# Autodesk Inventor assembly: PCBAssembly
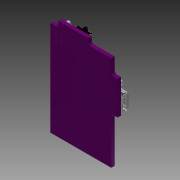
[picture p0: Inventor's stored thumbnail of the model, 180x180]
Saved by Autodesk Inventor 2015 SP2 (Build 190223200, 223)
## iProperties
Created: 2016-07-20
Part Number: PCBAssembly
Document SubType Name: Assembly
Designer: Iain
Author: Iain
## Documents named in this file (6)
- D:\Sit-To-Stand\BLEVibrator\Hardware\Case\PCBAssembly.iam
- D:\Sit-To-Stand\BLEVibrator\Hardware\Case\BarePCB.ipt
- D:\Sit-To-Stand\BLEVibrator\Hardware\Case\10118192C_USBHeader.ipt
- D:\Sit-To-Stand\BLEVibrator\Hardware\Case\RFDuino.ipt
- D:\Sit-To-Stand\BLEVibrator\Hardware\Case\SSSS810701_SlideSwitch.ipt
- D:\Sit-To-Stand\BLEVibrator\Hardware\Case\SM1204XXX_LED.ipt
## Components (6 placed, 5 different names)
1. BarePCB:1 — Mate:1, Mate:2, Flush:2, Flush:3, Mate:3, Mate:4, Flush:4, Flush:5, Flush:6, Mate:5, Mate:6, Flush:7, Flush:8, Flush:9, Flush:10
2. 10118192C_USBHeader:1 — Mate:3, Mate:4, Flush:4
3. RFDuino:1 — Mate:1, Flush:2, Flush:3
4. SSSS810701_SlideSwitch:1 — Mate:2, Flush:5, Flush:6
5. SM1204XXX_LED:1 — Mate:6, Flush:9, Flush:10
6. SM1204XXX_LED:2 — Mate:5, Flush:7, Flush:8
## Relationships (15: Flush 9, Mate 6)
- Mate:1: BarePCB:1 ↔ RFDuino:1
- Mate:2: BarePCB:1 ↔ SSSS810701_SlideSwitch:1
- Flush:2 (3.6 mm): BarePCB:1 ↔ RFDuino:1
- Flush:3 (2.2 mm): BarePCB:1 ↔ RFDuino:1
- Mate:3 (0.5 mm): BarePCB:1 ↔ 10118192C_USBHeader:1
- Mate:4 (-1.6 mm): BarePCB:1 ↔ 10118192C_USBHeader:1
- Flush:4: BarePCB:1 ↔ 10118192C_USBHeader:1
- Flush:5: BarePCB:1 ↔ SSSS810701_SlideSwitch:1
- Flush:6 (1.05 mm): BarePCB:1 ↔ SSSS810701_SlideSwitch:1
- Mate:5: BarePCB:1 ↔ SM1204XXX_LED:2
- Mate:6: BarePCB:1 ↔ SM1204XXX_LED:1
- Flush:7 (0.85 mm): BarePCB:1 ↔ SM1204XXX_LED:2
- Flush:8 (1 mm): BarePCB:1 ↔ SM1204XXX_LED:2
- Flush:9 (0.85 mm): BarePCB:1 ↔ SM1204XXX_LED:1
- Flush:10 (1.35 mm): BarePCB:1 ↔ SM1204XXX_LED:1
